# Autodesk Inventor assembly: Intake Prototypes
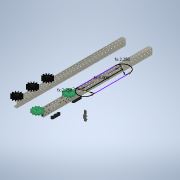
[picture p0: Inventor's stored thumbnail of the model, 180x180]
Saved by Autodesk Inventor 2020 (Build 240168000, 168)
## iProperties
Created: 2019-09-15
Part Number: Intake Prototypes
Document SubType Name: Assembly
Designer: Corey
Author: Corey
## Documents named in this file (7)
- C:\Users\Corey\Documents\Tower-Takeover-CAD\Intake Prototypes.iam
- C:\Users\Corey\Documents\Tower-Takeover-CAD\Parts\Structure\C-Channels\Aluminum\2-Wide\Aluminum C-Channel 1x2x1x35.ipt
- C:\Users\Corey\Documents\Tower-Takeover-CAD\Parts\Motion\Wheels & Rollers\Intake Roller.ipt
- C:\Users\Corey\Documents\Tower-Takeover-CAD\Parts\Motion\Sprockets\High Strength 12-tooth Sprocket.ipt
- C:\Users\Corey\Documents\Tower-Takeover-CAD\Parts\Motion\Chain & Tank Tread\Tank Tread Traction Link.ipt
- C:\Users\Corey\Documents\Tower-Takeover-CAD\Parts\Motion\Bearing Flat.ipt
- C:\Users\Corey\Documents\Tower-Takeover-CAD\Chain Sketch for Intake.ipt
## Components (17 placed, 6 different names)
1. Aluminum C-Channel 1x2x1x35:1
2. Intake Roller:1
3. Intake Roller:2
4. Intake Roller:3
5. Aluminum C-Channel 1x2x1x35:2 — Mate:1, Insert:1, Insert:2, Mate:2, Insert:3, Insert:4, Mate:3, Mate:4, Insert:5, Insert:6, Insert:7, Insert:8
6. High Strength 12-tooth Sprocket:1
7. High Strength 12-tooth Sprocket:2
8. Tank Tread Traction Link:1
9. Bearing Flat:1 — Mate:1, Insert:1, Insert:2
10. Bearing Flat:2 — Mate:3, Insert:5, Insert:6
11. Bearing Flat:3 — Mate:2, Insert:3, Insert:4
12. Bearing Flat:4
13. Bearing Flat:5 — Mate:4, Insert:7, Insert:8
14. Bearing Flat:6
15. Bearing Flat:7
16. Bearing Flat:8
17. Chain Sketch for Intake:1
## Relationships (12: Insert 8, Mate 4)
- Mate:1: Aluminum C-Channel 1x2x1x35:2 ↔ Bearing Flat:1
- Insert:1: Aluminum C-Channel 1x2x1x35:2 ↔ Bearing Flat:1
- Insert:2: Aluminum C-Channel 1x2x1x35:2 ↔ Bearing Flat:1
- Mate:2: Aluminum C-Channel 1x2x1x35:2 ↔ Bearing Flat:3
- Insert:3: Aluminum C-Channel 1x2x1x35:2 ↔ Bearing Flat:3
- Insert:4: Aluminum C-Channel 1x2x1x35:2 ↔ Bearing Flat:3
- Mate:3: Aluminum C-Channel 1x2x1x35:2 ↔ Bearing Flat:2
- Mate:4: Aluminum C-Channel 1x2x1x35:2 ↔ Bearing Flat:5
- Insert:5: Aluminum C-Channel 1x2x1x35:2 ↔ Bearing Flat:2
- Insert:6: Aluminum C-Channel 1x2x1x35:2 ↔ Bearing Flat:2
- Insert:7: Aluminum C-Channel 1x2x1x35:2 ↔ Bearing Flat:5
- Insert:8: Aluminum C-Channel 1x2x1x35:2 ↔ Bearing Flat:5
